# Autodesk Inventor assembly: Ellbow
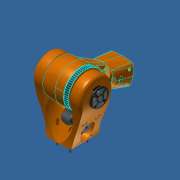
[picture p0: Inventor's stored thumbnail of the model, 180x180]
Saved by Autodesk Inventor 2014 SP2 (Build 180246200, 246)
## iProperties
Created: 2015-02-01
Part Number: Ellbow
Document SubType Name: Assembly
Designer: 4ndreas
Author: 4ndreas
## Documents named in this file (22)
- C:\Users\4ndreas\Documents\Inventor\RobotARM v2\v3\Ellbow.iam
- C:\Users\4ndreas\Documents\Inventor\RobotARM v2\v3\Ellbow_bearing_Motor.ipt
- C:\Users\4ndreas\Documents\Inventor\RobotARM v2\v3\Ellbow\Konstruktions-Assistent\Übertragung des Zahnriemens1.iam
- C:\Users\4ndreas\Documents\Inventor\RobotARM v2\v3\Conrad Motor.ipt
- C:\Users\4ndreas\Documents\Inventor\RobotARM v2\v2\elbow.iam
- C:\Users\4ndreas\Documents\Inventor\RobotARM v2\v3\EllbowMotorMount.ipt
- C:\Users\4ndreas\Documents\Inventor\Content Center Files\R2014\de-DE\DIN 9021\DIN 9021 - 4,3.ipt
- C:\Users\4ndreas\Documents\Inventor\Content Center Files\R2014\de-DE\DIN 125-1  A\DIN 125 - A 4,3.ipt
- C:\Users\4ndreas\Documents\Inventor\Content Center Files\R2014\de-DE\DIN 985\DIN 985 - M4.ipt
- C:\Users\4ndreas\Documents\Inventor\Content Center Files\R2014\de-DE\DIN BEARING(1)\DIN 625 SKF - SKF 624.ipt
- C:\Users\4ndreas\Documents\Inventor\RobotARM v2\v3\clamp.ipt
- C:\Users\4ndreas\Documents\Inventor\Content Center Files\R2014\de-DE\DIN 912\DIN 912 - M4 x 0,7 x 35 x 20.ipt
- C:\Users\4ndreas\Documents\Inventor\Content Center Files\R2014\de-DE\DIN 912\DIN 912 - M3 x 0,5 x 8 x 6,75.ipt
- C:\Users\4ndreas\Documents\Inventor\Content Center Files\R2014\de-DE\DIN 934\DIN 934 - M4 x 0,7.ipt
- C:\Users\4ndreas\Documents\Inventor\Content Center Files\R2014\de-DE\DIN 912\DIN 912 - M4 x 0,7 x 25 x 23,25.ipt
- C:\Users\4ndreas\Documents\Inventor\Content Center Files\R2014\de-DE\DIN 912\DIN 912 - M4 x 0,7 x 40 x 20.ipt
- C:\Users\4ndreas\Documents\Inventor\Content Center Files\R2014\de-DE\DIN BEARING(1)\DIN 625 SKF - SKF 608.ipt
- C:\Users\4ndreas\Documents\Inventor\Content Center Files\R2014\de-DE\DIN 931-1\DIN 931-1 - M8 x 60.ipt
- C:\Users\4ndreas\Documents\Inventor\RobotARM v2\v2\M8_encoderMagnet.ipt
- C:\Users\4ndreas\Documents\Inventor\RobotARM v2\v2\Magnet.ipt
- C:\Users\4ndreas\Documents\Inventor\RobotARM v2\v2\encoder.iam
- C:\Users\4ndreas\Documents\Inventor\RobotARM v2\Nema17_GearedStepper.ipt
## Components (51 placed, 21 different names)
1. Ellbow_bearing_Motor:1 — Passend:1, Passend:2, Winkel:1, Passend:6, Passend:7, Passend:10, Passend:13, Passend:25, Passend:72, Passend:73, Passend:74, Passend:75, Passend:76, Passend:77, Passend:78, Passend:79, Passend:80, Passend:81, Passend:82, Passend:83, Passend:84, Passend:85, Passend:86, Passend:87, Passend:88, Passend:89, Passend:90, Passend:91, Passend:101, Passend:103, Winkel:2
2. Übertragung des Zahnriemens:1 [sub-assembly] — Passend:4, Passend:5, Passend:11, Passend:22, Passend:56
3. Conrad Motor:1 — Passend:4, Passend:5, Fluchtend:1, Passend:104
4. elbow:1 [sub-assembly] — Passend:6, Passend:7
5. EllbowMotorMount:1 — Passend:58, Passend:59, Passend:60, Passend:61, Passend:62, Passend:63, Passend:64, Passend:65, Passend:66, Passend:67, Passend:105
6. DIN 912 - ersetzt durch DIN EN ISO 4762 M4 x 35:2 — Passend:8, Passend:9, Passend:11, Passend:12, Passend:14, Passend:16, Passend:17, Passend:18, Passend:45, Passend:48, Passend:50, Passend:52, Passend:55
7. DIN 9021 4,3:1 — Passend:12, Passend:13, Passend:15, Fluchtend:2
8. DIN 125-1 A A 4,3:1 — Passend:8, Passend:9, Passend:10
9. DIN 985 - ersetzt durch DIN EN ISO 10511 M4:1 — Passend:16, Passend:47
10. DIN 125-1 A A 4,3:2 — Passend:14, Passend:15, Passend:54
11. DIN 625 SKF 624:1 — Passend:18, Passend:19, Passend:51
12. DIN 625 SKF 624:2 — Passend:17, Passend:19, Passend:49
13. DIN 912 - ersetzt durch DIN EN ISO 4762 M4 x 35:1 — Passend:22, Passend:23, Passend:24, Passend:26, Passend:27, Passend:28, Passend:31, Passend:32, Passend:35, Passend:39, Passend:42
14. DIN 125-1 A A 4,3:3 — Passend:23, Passend:24, Passend:25
15. DIN 985 - ersetzt durch DIN EN ISO 10511 M4:2 — Passend:26, Passend:44
16. DIN 625 SKF 624:3 — Passend:27, Passend:29, Passend:40
17. DIN 625 SKF 624:4 — Passend:28, Passend:29, Passend:38
18. DIN 9021 4,3:2 — Passend:32, Passend:33, Fluchtend:2
19. DIN 125-1 A A 4,3:4 — Passend:31, Passend:33, Passend:36
20. clamp:1 — Passend:41, Passend:43, Passend:46, Passend:55, Passend:56, Passend:57
21. DIN 125-1 A A 4,3:5 — Passend:34, Passend:37, Passend:38
22. DIN 125-1 A A 4,3:6 — Passend:34, Passend:35, Passend:36, Passend:37
23. DIN 125-1 A A 4,3:7 — Passend:39, Passend:40, Passend:41
24. DIN 9021 4,3:3 — Passend:42, Passend:43, Passend:44
25. DIN 9021 4,3:4 — Passend:45, Passend:46, Passend:47
26. DIN 125-1 A A 4,3:8 — Passend:50, Passend:51, Passend:53
27. DIN 125-1 A A 4,3:9 — Passend:48, Passend:49
28. DIN 125-1 A A 4,3:10 — Passend:52, Passend:53, Passend:54
29. DIN 912 - ersetzt durch DIN EN ISO 4762 M3 x 8:1 — Passend:59, Passend:62
30. DIN 912 - ersetzt durch DIN EN ISO 4762 M3 x 8:2 — Passend:60, Passend:63
31. DIN 912 - ersetzt durch DIN EN ISO 4762 M3 x 8:3 — Passend:58, Passend:61
32. DIN 934 - ersetzt durch DIN EN 24032/28673/28674 M4:1 — Passend:64, Passend:66
33. DIN 934 - ersetzt durch DIN EN 24032/28673/28674 M4:2 — Passend:65, Passend:67
34. DIN 912 - ersetzt durch DIN EN ISO 4762 M4 x 25:1 — Passend:69, Passend:71, Passend:74
35. DIN 912 - ersetzt durch DIN EN ISO 4762 M4 x 25:2 — Passend:68, Passend:70, Passend:75
36. DIN 125-1 A A 4,3:11 — Passend:68, Passend:70, Passend:72
37. DIN 125-1 A A 4,3:12 — Passend:69, Passend:71, Passend:73
38. DIN 912 - ersetzt durch DIN EN ISO 4762 M4 x 40:1 — Passend:79, Passend:81
39. DIN 912 - ersetzt durch DIN EN ISO 4762 M4 x 40:2 — Passend:78, Passend:80
40. DIN 912 - ersetzt durch DIN EN ISO 4762 M4 x 40:3 — Passend:77, Passend:82
41. DIN 912 - ersetzt durch DIN EN ISO 4762 M4 x 40:4 — Passend:76, Passend:83
42. DIN 625 SKF 608:1 — Passend:84, Passend:88, Passend:92, Passend:95
43. DIN 625 SKF 608:2 — Passend:85, Passend:91, Passend:93, Passend:94
44. DIN 625 SKF 608:3 — Passend:86, Passend:89
45. DIN 625 SKF 608:4 — Passend:87, Passend:90
46. DIN 931-1 - ersetzt durch DIN EN 24014 M8 x 60:1 — Passend:92, Passend:95, Passend:96, Passend:97, Passend:98
47. DIN 931-1 - ersetzt durch DIN EN 24014 M8 x 60:2 — Passend:93, Passend:94
48. M8_encoderMagnet:1 — Passend:96, Passend:97, Passend:98, Passend:99, Passend:100
49. Magnet:1 — Passend:99, Passend:100, Passend:102
50. encoder:1 [sub-assembly] — Passend:101, Passend:102, Passend:103
51. Nema17_GearedStepper:1 — Passend:104, Passend:105, Winkel:2
## Relationships (106: Mate 102, Angle 2, Flush 2)
- Passend:1 [Mate]: Ellbow_bearing_Motor:1
- Passend:2 [Mate]: Ellbow_bearing_Motor:1
- Passend:3 [Mate]
- Winkel:1 [Angle] (90 deg): Ellbow_bearing_Motor:1
- Passend:4 [Mate]: Übertragung des Zahnriemens:1 ↔ Conrad Motor:1
- Passend:5 [Mate] (1 mm): Übertragung des Zahnriemens:1 ↔ Conrad Motor:1
- Fluchtend:1 [Flush]: Conrad Motor:1
- Passend:6 [Mate]: Ellbow_bearing_Motor:1 ↔ elbow:1
- Passend:7 [Mate] (0.5 mm): Ellbow_bearing_Motor:1 ↔ elbow:1
- Passend:8 [Mate]: DIN 912 - ersetzt durch DIN EN ISO 4762 M4 x 35:2 ↔ DIN 125-1 A A 4,3:1
- Passend:9 [Mate]: DIN 912 - ersetzt durch DIN EN ISO 4762 M4 x 35:2 ↔ DIN 125-1 A A 4,3:1
- Passend:10 [Mate]: Ellbow_bearing_Motor:1 ↔ DIN 125-1 A A 4,3:1
- Passend:11 [Mate]: Übertragung des Zahnriemens:1 ↔ DIN 912 - ersetzt durch DIN EN ISO 4762 M4 x 35:2
- Passend:12 [Mate]: DIN 912 - ersetzt durch DIN EN ISO 4762 M4 x 35:2 ↔ DIN 9021 4,3:1
- Passend:13 [Mate]: Ellbow_bearing_Motor:1 ↔ DIN 9021 4,3:1
- Passend:14 [Mate]: DIN 912 - ersetzt durch DIN EN ISO 4762 M4 x 35:2 ↔ DIN 125-1 A A 4,3:2
- Passend:15 [Mate]: DIN 9021 4,3:1 ↔ DIN 125-1 A A 4,3:2
- Passend:16 [Mate]: DIN 912 - ersetzt durch DIN EN ISO 4762 M4 x 35:2 ↔ DIN 985 - ersetzt durch DIN EN ISO 10511 M4:1
- Passend:17 [Mate]: DIN 912 - ersetzt durch DIN EN ISO 4762 M4 x 35:2 ↔ DIN 625 SKF 624:2
- Passend:18 [Mate]: DIN 912 - ersetzt durch DIN EN ISO 4762 M4 x 35:2 ↔ DIN 625 SKF 624:1
- Passend:19 [Mate]: DIN 625 SKF 624:1 ↔ DIN 625 SKF 624:2
- Passend:22 [Mate]: Übertragung des Zahnriemens:1 ↔ DIN 912 - ersetzt durch DIN EN ISO 4762 M4 x 35:1
- Passend:23 [Mate]: DIN 912 - ersetzt durch DIN EN ISO 4762 M4 x 35:1 ↔ DIN 125-1 A A 4,3:3
- Passend:24 [Mate]: DIN 912 - ersetzt durch DIN EN ISO 4762 M4 x 35:1 ↔ DIN 125-1 A A 4,3:3
- Passend:25 [Mate]: Ellbow_bearing_Motor:1 ↔ DIN 125-1 A A 4,3:3
- Passend:26 [Mate]: DIN 912 - ersetzt durch DIN EN ISO 4762 M4 x 35:1 ↔ DIN 985 - ersetzt durch DIN EN ISO 10511 M4:2
- Passend:27 [Mate]: DIN 912 - ersetzt durch DIN EN ISO 4762 M4 x 35:1 ↔ DIN 625 SKF 624:3
- Passend:28 [Mate]: DIN 912 - ersetzt durch DIN EN ISO 4762 M4 x 35:1 ↔ DIN 625 SKF 624:4
- Passend:29 [Mate]: DIN 625 SKF 624:3 ↔ DIN 625 SKF 624:4
- Passend:31 [Mate]: DIN 912 - ersetzt durch DIN EN ISO 4762 M4 x 35:1 ↔ DIN 125-1 A A 4,3:4
- Passend:32 [Mate]: DIN 912 - ersetzt durch DIN EN ISO 4762 M4 x 35:1 ↔ DIN 9021 4,3:2
- Passend:33 [Mate]: DIN 9021 4,3:2 ↔ DIN 125-1 A A 4,3:4
- Fluchtend:2 [Flush]: DIN 9021 4,3:1 ↔ DIN 9021 4,3:2
- Passend:34 [Mate]: DIN 125-1 A A 4,3:5 ↔ DIN 125-1 A A 4,3:6
- Passend:35 [Mate]: DIN 912 - ersetzt durch DIN EN ISO 4762 M4 x 35:1 ↔ DIN 125-1 A A 4,3:6
- Passend:36 [Mate]: DIN 125-1 A A 4,3:4 ↔ DIN 125-1 A A 4,3:6
- Passend:37 [Mate]: DIN 125-1 A A 4,3:5 ↔ DIN 125-1 A A 4,3:6
- Passend:38 [Mate]: DIN 625 SKF 624:4 ↔ DIN 125-1 A A 4,3:5
- Passend:39 [Mate]: DIN 912 - ersetzt durch DIN EN ISO 4762 M4 x 35:1 ↔ DIN 125-1 A A 4,3:7
- Passend:40 [Mate]: DIN 625 SKF 624:3 ↔ DIN 125-1 A A 4,3:7
- Passend:41 [Mate]: clamp:1 ↔ DIN 125-1 A A 4,3:7
- Passend:42 [Mate]: DIN 912 - ersetzt durch DIN EN ISO 4762 M4 x 35:1 ↔ DIN 9021 4,3:3
- Passend:43 [Mate]: clamp:1 ↔ DIN 9021 4,3:3
- Passend:44 [Mate]: DIN 985 - ersetzt durch DIN EN ISO 10511 M4:2 ↔ DIN 9021 4,3:3
- Passend:45 [Mate]: DIN 912 - ersetzt durch DIN EN ISO 4762 M4 x 35:2 ↔ DIN 9021 4,3:4
- Passend:46 [Mate]: clamp:1 ↔ DIN 9021 4,3:4
- Passend:47 [Mate]: DIN 985 - ersetzt durch DIN EN ISO 10511 M4:1 ↔ DIN 9021 4,3:4
- Passend:48 [Mate]: DIN 912 - ersetzt durch DIN EN ISO 4762 M4 x 35:2 ↔ DIN 125-1 A A 4,3:9
- Passend:49 [Mate]: DIN 625 SKF 624:2 ↔ DIN 125-1 A A 4,3:9
- Passend:50 [Mate]: DIN 912 - ersetzt durch DIN EN ISO 4762 M4 x 35:2 ↔ DIN 125-1 A A 4,3:8
- Passend:51 [Mate]: DIN 625 SKF 624:1 ↔ DIN 125-1 A A 4,3:8
- Passend:52 [Mate]: DIN 912 - ersetzt durch DIN EN ISO 4762 M4 x 35:2 ↔ DIN 125-1 A A 4,3:10
- Passend:53 [Mate]: DIN 125-1 A A 4,3:8 ↔ DIN 125-1 A A 4,3:10
- Passend:54 [Mate]: DIN 125-1 A A 4,3:2 ↔ DIN 125-1 A A 4,3:10
- Passend:55 [Mate]: DIN 912 - ersetzt durch DIN EN ISO 4762 M4 x 35:2 ↔ clamp:1
- Passend:56 [Mate]: Übertragung des Zahnriemens:1 ↔ clamp:1
- Passend:57 [Mate]: clamp:1
- Passend:58 [Mate]: EllbowMotorMount:1 ↔ DIN 912 - ersetzt durch DIN EN ISO 4762 M3 x 8:3
- Passend:59 [Mate]: EllbowMotorMount:1 ↔ DIN 912 - ersetzt durch DIN EN ISO 4762 M3 x 8:1
- Passend:60 [Mate]: EllbowMotorMount:1 ↔ DIN 912 - ersetzt durch DIN EN ISO 4762 M3 x 8:2
- Passend:61 [Mate]: EllbowMotorMount:1 ↔ DIN 912 - ersetzt durch DIN EN ISO 4762 M3 x 8:3
- Passend:62 [Mate]: EllbowMotorMount:1 ↔ DIN 912 - ersetzt durch DIN EN ISO 4762 M3 x 8:1
- Passend:63 [Mate]: EllbowMotorMount:1 ↔ DIN 912 - ersetzt durch DIN EN ISO 4762 M3 x 8:2
- Passend:64 [Mate]: EllbowMotorMount:1 ↔ DIN 934 - ersetzt durch DIN EN 24032/28673/28674 M4:1
- Passend:65 [Mate]: EllbowMotorMount:1 ↔ DIN 934 - ersetzt durch DIN EN 24032/28673/28674 M4:2
- Passend:66 [Mate]: EllbowMotorMount:1 ↔ DIN 934 - ersetzt durch DIN EN 24032/28673/28674 M4:1
- Passend:67 [Mate]: EllbowMotorMount:1 ↔ DIN 934 - ersetzt durch DIN EN 24032/28673/28674 M4:2
- Passend:68 [Mate]: DIN 912 - ersetzt durch DIN EN ISO 4762 M4 x 25:2 ↔ DIN 125-1 A A 4,3:11
- Passend:69 [Mate]: DIN 912 - ersetzt durch DIN EN ISO 4762 M4 x 25:1 ↔ DIN 125-1 A A 4,3:12
- Passend:70 [Mate]: DIN 912 - ersetzt durch DIN EN ISO 4762 M4 x 25:2 ↔ DIN 125-1 A A 4,3:11
- Passend:71 [Mate]: DIN 912 - ersetzt durch DIN EN ISO 4762 M4 x 25:1 ↔ DIN 125-1 A A 4,3:12
- Passend:72 [Mate]: Ellbow_bearing_Motor:1 ↔ DIN 125-1 A A 4,3:11
- Passend:73 [Mate]: Ellbow_bearing_Motor:1 ↔ DIN 125-1 A A 4,3:12
- Passend:74 [Mate]: Ellbow_bearing_Motor:1 ↔ DIN 912 - ersetzt durch DIN EN ISO 4762 M4 x 25:1
- Passend:75 [Mate]: Ellbow_bearing_Motor:1 ↔ DIN 912 - ersetzt durch DIN EN ISO 4762 M4 x 25:2
- Passend:76 [Mate]: Ellbow_bearing_Motor:1 ↔ DIN 912 - ersetzt durch DIN EN ISO 4762 M4 x 40:4
- Passend:77 [Mate]: Ellbow_bearing_Motor:1 ↔ DIN 912 - ersetzt durch DIN EN ISO 4762 M4 x 40:3
- Passend:78 [Mate]: Ellbow_bearing_Motor:1 ↔ DIN 912 - ersetzt durch DIN EN ISO 4762 M4 x 40:2
- Passend:79 [Mate]: Ellbow_bearing_Motor:1 ↔ DIN 912 - ersetzt durch DIN EN ISO 4762 M4 x 40:1
- Passend:80 [Mate]: Ellbow_bearing_Motor:1 ↔ DIN 912 - ersetzt durch DIN EN ISO 4762 M4 x 40:2
- Passend:81 [Mate]: Ellbow_bearing_Motor:1 ↔ DIN 912 - ersetzt durch DIN EN ISO 4762 M4 x 40:1
- Passend:82 [Mate]: Ellbow_bearing_Motor:1 ↔ DIN 912 - ersetzt durch DIN EN ISO 4762 M4 x 40:3
- Passend:83 [Mate]: Ellbow_bearing_Motor:1 ↔ DIN 912 - ersetzt durch DIN EN ISO 4762 M4 x 40:4
- Passend:84 [Mate]: Ellbow_bearing_Motor:1 ↔ DIN 625 SKF 608:1
- Passend:85 [Mate]: Ellbow_bearing_Motor:1 ↔ DIN 625 SKF 608:2
- Passend:86 [Mate]: Ellbow_bearing_Motor:1 ↔ DIN 625 SKF 608:3
- Passend:87 [Mate]: Ellbow_bearing_Motor:1 ↔ DIN 625 SKF 608:4
- Passend:88 [Mate]: Ellbow_bearing_Motor:1 ↔ DIN 625 SKF 608:1
- Passend:89 [Mate]: Ellbow_bearing_Motor:1 ↔ DIN 625 SKF 608:3
- Passend:90 [Mate]: Ellbow_bearing_Motor:1 ↔ DIN 625 SKF 608:4
- Passend:91 [Mate]: Ellbow_bearing_Motor:1 ↔ DIN 625 SKF 608:2
- Passend:92 [Mate]: DIN 625 SKF 608:1 ↔ DIN 931-1 - ersetzt durch DIN EN 24014 M8 x 60:1
- Passend:93 [Mate]: DIN 625 SKF 608:2 ↔ DIN 931-1 - ersetzt durch DIN EN 24014 M8 x 60:2
- Passend:94 [Mate]: DIN 625 SKF 608:2 ↔ DIN 931-1 - ersetzt durch DIN EN 24014 M8 x 60:2
- Passend:95 [Mate]: DIN 625 SKF 608:1 ↔ DIN 931-1 - ersetzt durch DIN EN 24014 M8 x 60:1
- Passend:96 [Mate]: DIN 931-1 - ersetzt durch DIN EN 24014 M8 x 60:1 ↔ M8_encoderMagnet:1
- Passend:97 [Mate]: DIN 931-1 - ersetzt durch DIN EN 24014 M8 x 60:1 ↔ M8_encoderMagnet:1
- Passend:98 [Mate]: DIN 931-1 - ersetzt durch DIN EN 24014 M8 x 60:1 ↔ M8_encoderMagnet:1
- Passend:99 [Mate]: M8_encoderMagnet:1 ↔ Magnet:1
- Passend:100 [Mate]: M8_encoderMagnet:1 ↔ Magnet:1
- Passend:101 [Mate]: Ellbow_bearing_Motor:1 ↔ encoder:1
- Passend:102 [Mate] (1 mm): Magnet:1 ↔ encoder:1
- Passend:103 [Mate]: Ellbow_bearing_Motor:1 ↔ encoder:1
- Passend:104 [Mate]: Conrad Motor:1 ↔ Nema17_GearedStepper:1
- Passend:105 [Mate]: EllbowMotorMount:1 ↔ Nema17_GearedStepper:1
- Winkel:2 [Angle] (0 deg): Ellbow_bearing_Motor:1 ↔ Nema17_GearedStepper:1
